# Autodesk Inventor assembly: MotorAss
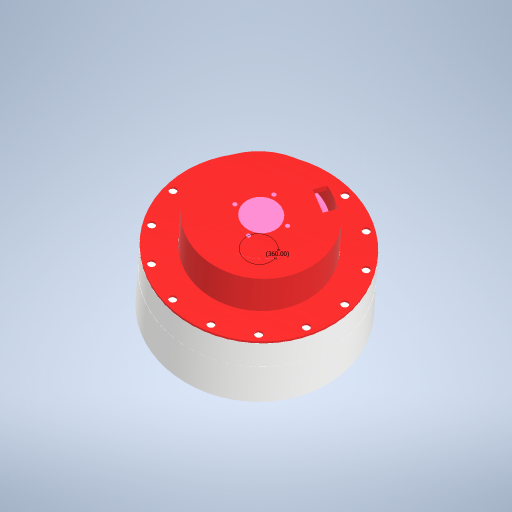
[picture p0: Inventor's stored thumbnail of the model, 512x512]
Saved by Autodesk Inventor 2023 (Build 270158000, 158)
## iProperties
Created: 2023-03-29
Part Number: MotorAss
Document SubType Name: Assembly
Designer: Charles Kelly
Author: Charles Kelly
## Documents named in this file (5)
- C:\Users\Charles Kelly\Documents\Inventor\Robtooc\Apparatus\THE ARM\MotorAss.iam
- C:\Users\Charles Kelly\Documents\Inventor\Robtooc\Apparatus\THE ARM\Wrist\EAGLE POWER 8308.ipt
- C:\Users\Charles Kelly\Documents\Inventor\Robtooc\Apparatus\THE ARM\EaglePowerCycDriveAdaptor.ipt
- C:\Users\Charles Kelly\Documents\Inventor\Robtooc\Apparatus\Cycloidal Drive\Drive.iam
- C:\Users\Charles Kelly\Documents\Inventor\Robtooc\Apparatus\THE ARM\MotorCycDriveMount.ipt
## Components (4 placed, 4 different names)
1. EAGLE POWER 8308:1 — Rotational:1
2. EaglePowerCycDriveAdaptor:1 — Rotational:1, Cylindrical:1, Rotational:2
3. Drive:1 [sub-assembly] — Cylindrical:1, Rotational:2, Rotational:3
4. MotorCycDriveMount:1 — Rotational:3
## Relationships (4: RevoluteJoint 3, CylindricalJoint 1)
- Rotational:1 [RevoluteJoint]: EAGLE POWER 8308:1 ↔ EaglePowerCycDriveAdaptor:1
- Cylindrical:1: EaglePowerCycDriveAdaptor:1 ↔ Drive:1
- Rotational:2 [RevoluteJoint]: EaglePowerCycDriveAdaptor:1 ↔ Drive:1
- Rotational:3 [RevoluteJoint]: Drive:1 ↔ MotorCycDriveMount:1
